# Autodesk Inventor assembly: CONVEYOR-01
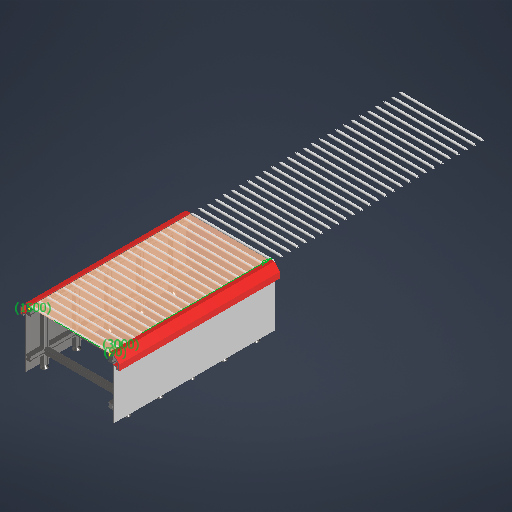
[picture p0: Inventor's stored thumbnail of the model, 512x512]
Saved by Autodesk Inventor 2025 (Build 290162000, 162)
## iProperties
RuleStatus: InUse
Created: 2024-05-06
Part Number: CONVEYOR-01
Document SubType Name: Assembly
Designer: zulet
Author: zulet
rollerSeparation: 90,000 mm
conveyorLength: 3000,000 mm
rollerLength: 1500,000 mm
## Documents named in this file (8)
- D:\UNAL\2024-1S\APM\Digital Factory\Conveyor System\CONVEYOR\CONVEYOR-1500x3000x1135.iam
- D:\UNAL\2024-1S\APM\Digital Factory\Conveyor System\CONVEYOR STRUCTURE.ipt
- D:\UNAL\2024-1S\APM\Digital Factory\Conveyor System\CONVEYOR ROLLER.ipt
- D:\UNAL\2024-1S\APM\Digital Factory\Conveyor System\CONVEYOR SURFACE.ipt
- D:\UNAL\2024-1S\APM\Digital Factory\Conveyor System\CONVEYOR STRUCTURE\CONVEYOR STRUCTURE-04.ipt
- D:\UNAL\2024-1S\APM\Digital Factory\Conveyor System\CONVEYOR ROLLER\CR-1500.ipt
- D:\UNAL\2024-1S\APM\Digital Factory\Conveyor System\CONVEYOR SURFACE\CONVEYOR SURFACE-1500x3000.ipt
- D:\UNAL\2024-1S\APM\Digital Factory\Conveyor System\CONVEYOR.iam
## Components (49 placed, 3 different names)
1. CONVEYOR STRUCTURE-04:1 — Mate:1, Mate:2, Rigid:1
2. CONVEYOR SURFACE-1500x3000:1 — Rigid:1
3. CR-1500:1 — Mate:1, Mate:2
4. CR-1500:2
5. CR-1500:3
6. CR-1500:4
7. CR-1500:5
8. CR-1500:6
9. CR-1500:7
10. CR-1500:8
11. CR-1500:9
12. CR-1500:10
13. CR-1500:11
14. CR-1500:12
15. CR-1500:13
16. CR-1500:14
17. CR-1500:15
18. CR-1500:16
19. CR-1500:17
20. CR-1500:18
21. CR-1500:19
22. CR-1500:20
23. CR-1500:21
24. CR-1500:22
25. CR-1500:23
26. CR-1500:24
27. CR-1500:25
28. CR-1500:26
29. CR-1500:27
30. CR-1500:28
31. CR-1500:29
32. CR-1500:30
33. CR-1500:31
34. CR-1500:32
35. CR-1500:33
36. CR-1500:34
37. CR-1500:35
38. CR-1500:36
39. CR-1500:37
40. CR-1500:38
41. CR-1500:40
42. CR-1500:41
43. CR-1500:42
44. CR-1500:43
45. CR-1500:44
46. CR-1500:45
47. CR-1500:46
48. CR-1500:47
49. CR-1500:48
## Component patterns: (47 elements, first: CR-1500:1)
## Relationships (3: Mate 2, WeldJoint 1)
- Mate:1: CONVEYOR STRUCTURE-04:1 ↔ CR-1500:1
- Mate:2: CONVEYOR STRUCTURE-04:1 ↔ CR-1500:1
- Rigid:1 [WeldJoint]: CONVEYOR STRUCTURE-04:1 ↔ CONVEYOR SURFACE-1500x3000:1
